# Autodesk Inventor assembly: Chassis
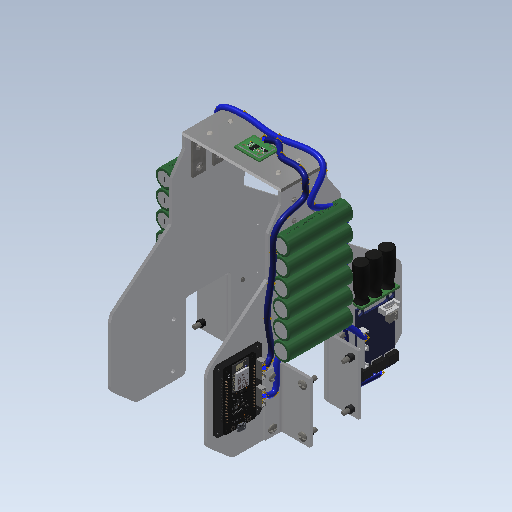
[picture p0: Inventor's stored thumbnail of the model, 512x512]
Saved by Autodesk Inventor 2020 (Build 240168000, 168)
## iProperties
Created: 2019-05-15
Part Number: Chassis
Document SubType Name: Assembly
Designer: Administrator
Mass: 571.597 g
Surface Area: 1580.61 cm^2
Volume: 207.619 cm^3
Density: 2.75311 g/cm^3
Title: Chassis
Author: Administrator
## Documents named in this file (25)
- C:\Users\chitl\Desktop\OneWheel\Wheel Assembled\Chassis\Chassis.iam
- C:\Users\chitl\Desktop\OneWheel\Wheel Assembled\Chassis\Fastners\8-32 Screw - 0.5 .ipt
- C:\Users\chitl\Desktop\OneWheel\Wheel Assembled\Chassis\Fastners\8-32 Screw 0.5.ipt
- C:\Users\chitl\Desktop\OneWheel\Wheel Assembled\Chassis\Fastners\8-32 Screw 0.25 (1).ipt
- C:\Users\chitl\Desktop\OneWheel\Wheel Assembled\Chassis\Fastners\8-32 Screw 0.25.ipt
- C:\Users\chitl\Desktop\OneWheel\Wheel Assembled\Chassis\Fastners\8-32 Scew 0.25.ipt
- C:\Users\chitl\Desktop\OneWheel\Wheel Assembled\Chassis\Fastners\8-32 Screw 0.5 (1).ipt
- C:\Users\chitl\Desktop\OneWheel\Wheel Assembled\Chassis\L-Braces\L-Brace (1).ipt
- C:\Users\chitl\Desktop\OneWheel\Wheel Assembled\Chassis\L-Braces\L-Brace.ipt
- C:\Users\chitl\Desktop\OneWheel\Wheel Assembled\Chassis\Fastners\8-32 Screw 0.5 .ipt
- C:\Users\chitl\Desktop\OneWheel\Wheel Assembled\Chassis\Fastners\8-32 Screw 0.25 .ipt
- C:\Users\chitl\Desktop\OneWheel\Wheel Assembled\Chassis\L-Braces\L-Brace (3).ipt
- C:\Users\chitl\Desktop\OneWheel\Wheel Assembled\Chassis\L-Braces\L-Brace (2).ipt
- C:\Users\chitl\Desktop\OneWheel\Wheel Assembled\Chassis\L-Braces\1556A42.ipt
- C:\Users\chitl\Desktop\OneWheel\Wheel Assembled\Chassis\Fastners\91500A190.ipt
- C:\Users\chitl\Desktop\OneWheel\Wheel Assembled\Chassis\L-Braces\1556A42(Mirror) (1).ipt
- C:\Users\chitl\Desktop\OneWheel\Wheel Assembled\Chassis\Fastners\91500A190(Mirror).ipt
- C:\Users\chitl\Desktop\OneWheel\Wheel Assembled\Chassis\Fastners\8-32 Screw 0.5 (1)(Mirror).ipt
- C:\Users\chitl\Desktop\OneWheel\Wheel Assembled\Chassis\Chassis.ipt
- C:\Users\chitl\Desktop\OneWheel\Wheel Assembled\Electronics\18650 Battery.ipt
- C:\Users\chitl\Desktop\OneWheel\Wheel Assembled\Electronics\MPU 9250.ipt
- C:\Users\chitl\Desktop\OneWheel\Wheel Assembled\Electronics\VESC.ipt
- C:\Users\chitl\Desktop\OneWheel\Wheel Assembled\Electronics\Controller_PCB.iam
- C:\Users\chitl\Desktop\OneWheel\Wheel Assembled\Chassis\Chassis\AIP\Tube and Pipe\Cable and Harness\Chassis.Harness2.iam
- C:\Users\chitl\Desktop\OneWheel\Wheel Assembled\Chassis\Misc\Bushing.ipt
## Components (53 placed, 24 different names)
1. 8-32 Screw - 0.5 :1
2. 8-32 Screw - 0.5 :2
3. 8-32 Screw 0.5:2
4. 8-32 Screw 0.25 (1):2
5. 8-32 Screw 0.25:2
6. 8-32 Screw 0.25 (1):1
7. 8-32 Scew 0.25:2
8. 8-32 Scew 0.25:1
9. 8-32 Screw 0.5:1
10. 8-32 Screw 0.25:1
11. 8-32 Screw 0.5 (1):1
12. 8-32 Screw 0.5 (1):2
13. L-Brace (1):1 — Rigid:3, Rigid:4
14. L-Brace:1 — Rigid:1, Rigid:2
15. 8-32 Screw 0.5 :2
16. 8-32 Screw 0.25 :2
17. 8-32 Screw 0.25 :1
18. 8-32 Screw 0.5 :1
19. L-Brace (3):1 — Rigid:7, Rigid:8
20. L-Brace (2):1 — Rigid:5, Rigid:6
21. 1556A42:1
22. 91500A190:1
23. 1556A42(Mirror) (1):1
24. 1556A42:2
25. 1556A42(Mirror) (1):2
26. 91500A190:2
27. 91500A190:4
28. 91500A190:5
29. 91500A190:3
30. 91500A190:6
31. 91500A190(Mirror):5
32. 91500A190(Mirror):2
33. 91500A190(Mirror):1
34. 91500A190(Mirror):3
35. 91500A190(Mirror):6
36. 91500A190(Mirror):4
37. 8-32 Screw 0.5 (1)(Mirror):1
38. 8-32 Screw 0.5 (1)(Mirror):2
39. Chassis — Mate:1, Mate:2, Mate:7
40. 18650 Battery:1 — Mate:3, Mate:4, Mate:5, Mate:6
41. 18650 Battery:2
42. MPU 9250:1 — Mate:1
43. VESC:1 — Mate:2
44. Controller_PCB:1 [sub-assembly] — Mate:7
45. Harness2 [sub-assembly]
46. Bushing:1 — Rigid:1
47. Bushing:2 — Rigid:2
48. Bushing:3 — Rigid:3
49. Bushing:4 — Rigid:4
50. Bushing:5 — Rigid:5
51. Bushing:6 — Rigid:6
52. Bushing:7 — Rigid:7
53. Bushing:8 — Rigid:8
## Relationships (15: WeldJoint 8, Mate 7)
- Mate:1: Chassis ↔ MPU 9250:1
- Mate:2: Chassis ↔ VESC:1
- Mate:3: 18650 Battery:1
- Mate:4: 18650 Battery:1
- Mate:5: 18650 Battery:1
- Mate:6: 18650 Battery:1
- Mate:7: Chassis ↔ Controller_PCB:1
- Rigid:1 [WeldJoint]: L-Brace:1 ↔ Bushing:1
- Rigid:2 [WeldJoint]: L-Brace:1 ↔ Bushing:2
- Rigid:3 [WeldJoint]: L-Brace (1):1 ↔ Bushing:3
- Rigid:4 [WeldJoint]: L-Brace (1):1 ↔ Bushing:4
- Rigid:5 [WeldJoint]: L-Brace (2):1 ↔ Bushing:5
- Rigid:6 [WeldJoint]: L-Brace (2):1 ↔ Bushing:6
- Rigid:7 [WeldJoint]: L-Brace (3):1 ↔ Bushing:7
- Rigid:8 [WeldJoint]: L-Brace (3):1 ↔ Bushing:8
